# Autodesk Inventor assembly: option 2 pit
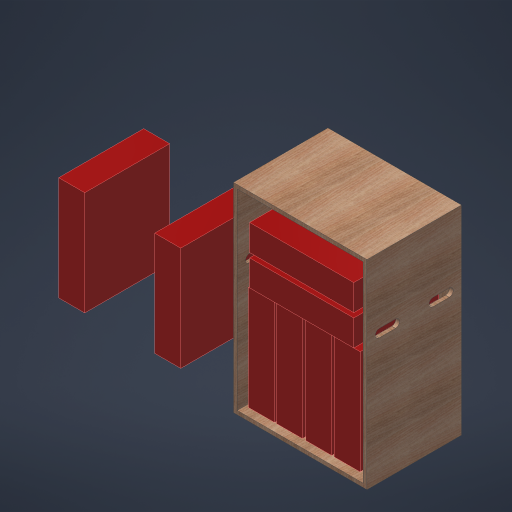
[picture p0: Inventor's stored thumbnail of the model, 512x512]
Saved by Autodesk Inventor 2023.4 (Build 274418000, 418)
## iProperties
Created: 2025-03-02
Part Number: option 2 pit
Document SubType Name: Assembly
Designer: brand
Author: brand
## Documents named in this file (3)
- C:\Users\brand\OneDrive\Documents\GitHub\robotics 23\2025-ReefScape---CAD\Pit\option 2 pit.iam
- C:\Users\brand\OneDrive\Documents\GitHub\robotics 23\2025-ReefScape---CAD\Pit\old battery cart.ipt
- C:\Users\brand\OneDrive\Documents\GitHub\robotics 23\2025-ReefScape---CAD\Pit\big craftsman.ipt
## Components (9 placed, 2 different names)
1. old battery cart:1 — Mate:2, Mate:3
2. big craftsman:1 — Flush:1, Flush:6, Mate:2, Mate:3
3. big craftsman:2 — Flush:1, Flush:2, Flush:6, Flush:7
4. big craftsman:3 — Flush:2, Flush:3, Flush:7, Flush:8
5. big craftsman:4 — Flush:3, Flush:4, Flush:8, Flush:9
6. big craftsman:5 — Flush:4, Flush:5, Flush:9, Flush:10
7. big craftsman:6 — Flush:5, Flush:10, Flush:11, Mate:4
8. big craftsman:7 — Flush:11, Mate:4, Flush:12, Flush:13
9. big craftsman:8 — Flush:12, Flush:13
## Relationships (16: Flush 13, Mate 3)
- Flush:1: big craftsman:1 ↔ big craftsman:2
- Flush:2: big craftsman:2 ↔ big craftsman:3
- Flush:3: big craftsman:3 ↔ big craftsman:4
- Flush:4: big craftsman:4 ↔ big craftsman:5
- Flush:5: big craftsman:5 ↔ big craftsman:6
- Flush:6: big craftsman:1 ↔ big craftsman:2
- Flush:7: big craftsman:2 ↔ big craftsman:3
- Flush:8: big craftsman:3 ↔ big craftsman:4
- Flush:9: big craftsman:4 ↔ big craftsman:5
- Flush:10: big craftsman:5 ↔ big craftsman:6
- Mate:2: old battery cart:1 ↔ big craftsman:1
- Mate:3: old battery cart:1 ↔ big craftsman:1
- Flush:11: big craftsman:6 ↔ big craftsman:7
- Mate:4: big craftsman:6 ↔ big craftsman:7
- Flush:12: big craftsman:7 ↔ big craftsman:8
- Flush:13: big craftsman:7 ↔ big craftsman:8
